# Autodesk Inventor assembly: MotorEsOrsoHajtas
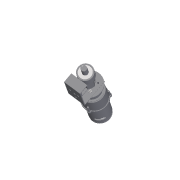
[picture p0: Inventor's stored thumbnail of the model, 180x180]
Saved by Autodesk Inventor 2015 SP1 (Build 190203100, 203)
## iProperties
Created: 2014-10-20
Part Number: MotorEsOrsoHajtas
Document SubType Name: Assembly
Designer: laca
Author: laca
## Documents named in this file (7)
- C:\Users\laca\Desktop\Allamvizsga\Invntor\RobotMechanikaForMAtlabVer2\MotorKerekHajtas.iam
- C:\Users\laca\Desktop\Allamvizsga\Invntor\RobotMechanikaForMAtlabVer2\MotorTartoElso.ipt
- C:\Users\laca\Desktop\Allamvizsga\Invntor\RobotMechanikaForMAtlabVer2\Csapagy6900.ipt
- C:\Users\laca\Desktop\Allamvizsga\Invntor\RobotMechanikaForMAtlabVer2\Biztositek15mm.ipt
- C:\Users\laca\Desktop\Allamvizsga\Invntor\RobotMechanikaForMAtlabVer2\Motor.iam
- C:\Users\laca\Desktop\Allamvizsga\Invntor\RobotMechanikaForMAtlabVer2\AnyaKicsiOldalso.ipt
- C:\Users\laca\Desktop\Allamvizsga\Invntor\RobotMechanikaForMAtlabVer2\MotorKerekHajtas\Design Accelerator\Bolted Connection2.iam
## Components (6 placed, 6 different names)
1. MotorTartoElso:1 — Rigid:1, Insert:5, Insert:6, Mate:1, Mate:2
2. Csapagy6900:2 — Rigid:1, Cylindrical:6
3. Biztositek15mm:2 — Cylindrical:4, Cylindrical:5, Flush:1
4. Motor:1 [sub-assembly] — Insert:5, Cylindrical:4, Insert:6
5. AnyaKicsiOldalso:1 — Cylindrical:5, Cylindrical:6, Flush:1
6. Bolted Connection:1 [sub-assembly] — Mate:1, Mate:2
## Relationships (9: CylindricalJoint 3, Insert 2, Mate 2, WeldJoint 1, Flush 1)
- Rigid:1 [WeldJoint]: MotorTartoElso:1 ↔ Csapagy6900:2
- Insert:5: MotorTartoElso:1 ↔ Motor:1
- Cylindrical:4: Biztositek15mm:2 ↔ Motor:1
- Insert:6: MotorTartoElso:1 ↔ Motor:1
- Cylindrical:5: Biztositek15mm:2 ↔ AnyaKicsiOldalso:1
- Cylindrical:6: Csapagy6900:2 ↔ AnyaKicsiOldalso:1
- Flush:1: Biztositek15mm:2 ↔ AnyaKicsiOldalso:1
- Mate:1: MotorTartoElso:1 ↔ Bolted Connection:1
- Mate:2: MotorTartoElso:1 ↔ Bolted Connection:1
